# Autodesk Inventor assembly: Колесо с осью
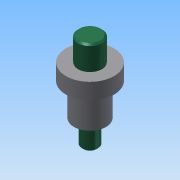
[picture p0: Inventor's stored thumbnail of the model, 180x180]
Saved by Autodesk Inventor 2013 (Build 170138000, 138)
## iProperties
Created: 2018-03-31
Part Number: Колесо с осью
Document SubType Name: Assembly
Designer: User
Author: User
## Documents named in this file (3)
- C:\Users\User\Documents\Пётр\Программирование\Мои сайты\Ris_Inventor\Колесо с осью.iam
- C:\Users\User\Documents\Пётр\Программирование\Мои сайты\Ris_Inventor\Колесо.ipt
- C:\Users\User\Documents\Пётр\Программирование\Мои сайты\Ris_Inventor\Ось.ipt
## Components (2 placed, 2 different names)
1. Колесо:1 — Заподлицо:1, Заподлицо:2, Заподлицо:3
2. Ось:1 — Заподлицо:1, Заподлицо:2, Заподлицо:3
## Relationships (3: Flush 3)
- Заподлицо:1 [Flush]: Колесо:1 ↔ Ось:1
- Заподлицо:2 [Flush]: Колесо:1 ↔ Ось:1
- Заподлицо:3 [Flush]: Колесо:1 ↔ Ось:1
